# Autodesk Inventor assembly: Wine Rack and Light Shelf Assembly
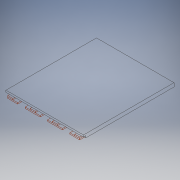
[picture p0: Inventor's stored thumbnail of the model, 180x180]
Saved by Autodesk Inventor 2016 (Build 200138000, 138)
## iProperties
Created: 2017-11-04
Part Number: Wine Rack and Light Shelf Assembly
Document SubType Name: Assembly
Designer: mathaetaes
Author: mathaetaes
## Documents named in this file (4)
- E:\Projects\3D Printer\printer projects\My Designs\Bar Cabinet 2.2.2018\Wine Rack and Light Shelf Assembly Right.iam
- E:\Projects\3D Printer\printer projects\My Designs\Bar Cabinet 2.2.2018\Horizontal Shelf with Lights.ipt
- E:\Projects\3D Printer\printer projects\My Designs\Bar Cabinet 2.2.2018\Wine Glass Rack Edge.iam
- E:\Projects\3D Printer\printer projects\My Designs\Bar Cabinet 2.2.2018\Wine Glass Rack Middle.iam
## Components (5 placed, 3 different names)
1. Horizontal Shelf with Lights:1 — Flush:4, Flush:5, Flush:6, Flush:7, Flush:8, Flush:9, Flush:10, Flush:11, Mate:1
2. Wine Glass Rack Middle:1 [sub-assembly] — Flush:2, Flush:3, Flush:6, Flush:10
3. Wine Glass Rack Edge:2 [sub-assembly] — Flush:1, Flush:4, Flush:8, Mate:1
4. Wine Glass Rack Middle:2 [sub-assembly] — Flush:1, Flush:2, Flush:5, Flush:9
5. Wine Glass Rack Edge:3 [sub-assembly] — Flush:3, Flush:7, Flush:11
## Relationships (12: Flush 11, Mate 1)
- Flush:1: Wine Glass Rack Edge:2 ↔ Wine Glass Rack Middle:2
- Flush:2: Wine Glass Rack Middle:1 ↔ Wine Glass Rack Middle:2
- Flush:3: Wine Glass Rack Middle:1 ↔ Wine Glass Rack Edge:3
- Flush:4: Horizontal Shelf with Lights:1 ↔ Wine Glass Rack Edge:2
- Flush:5: Horizontal Shelf with Lights:1 ↔ Wine Glass Rack Middle:2
- Flush:6: Horizontal Shelf with Lights:1 ↔ Wine Glass Rack Middle:1
- Flush:7: Horizontal Shelf with Lights:1 ↔ Wine Glass Rack Edge:3
- Flush:8: Horizontal Shelf with Lights:1 ↔ Wine Glass Rack Edge:2
- Flush:9: Horizontal Shelf with Lights:1 ↔ Wine Glass Rack Middle:2
- Flush:10: Horizontal Shelf with Lights:1 ↔ Wine Glass Rack Middle:1
- Flush:11: Horizontal Shelf with Lights:1 ↔ Wine Glass Rack Edge:3
- Mate:1: Horizontal Shelf with Lights:1 ↔ Wine Glass Rack Edge:2
